# Autodesk Inventor assembly: ArduinoProMicro
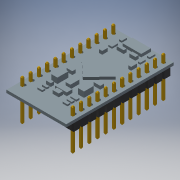
[picture p0: Inventor's stored thumbnail of the model, 180x180]
Saved by Autodesk Inventor 2018 (Build 220112000, 112)
## iProperties
Created: 2017-04-09
Part Number: ArduinoProMicro
Document SubType Name: Assembly
Designer: dkt01
Author: dkt01
## Documents named in this file (3)
- C:\Users\dktur\Dropbox\StackLightMonitor\CAD\ArduinoProMicro.iam
- C:\Users\dktur\Dropbox\StackLightMonitor\CAD\Arduino Pro Micro Sparkfun.ipt
- C:\Users\dktur\Dropbox\StackLightMonitor\CAD\MaleHeader-01.iam
## Components (3 placed, 2 different names)
1. Arduino Pro Micro Sparkfun:1 — Mate:1, Mate:2, Tangent:1, Tangent:2, Tangent:3, Tangent:4, Tangent:5, Tangent:6, Tangent:7, Tangent:8
2. MaleHeader-01:1 [sub-assembly] — Mate:1, Tangent:4, Tangent:5, Tangent:6, Tangent:8
3. MaleHeader-01:2 [sub-assembly] — Mate:2, Tangent:1, Tangent:2, Tangent:3, Tangent:7
## Relationships (10: Tangent 8, Mate 2)
- Mate:1: Arduino Pro Micro Sparkfun:1 ↔ MaleHeader-01:1
- Mate:2: Arduino Pro Micro Sparkfun:1 ↔ MaleHeader-01:2
- Tangent:1: Arduino Pro Micro Sparkfun:1 ↔ MaleHeader-01:2
- Tangent:2: Arduino Pro Micro Sparkfun:1 ↔ MaleHeader-01:2
- Tangent:3: Arduino Pro Micro Sparkfun:1 ↔ MaleHeader-01:2
- Tangent:4: Arduino Pro Micro Sparkfun:1 ↔ MaleHeader-01:1
- Tangent:5: Arduino Pro Micro Sparkfun:1 ↔ MaleHeader-01:1
- Tangent:6: Arduino Pro Micro Sparkfun:1 ↔ MaleHeader-01:1
- Tangent:7: Arduino Pro Micro Sparkfun:1 ↔ MaleHeader-01:2
- Tangent:8: Arduino Pro Micro Sparkfun:1 ↔ MaleHeader-01:1
